# Autodesk Inventor assembly: ArmTrussMIR
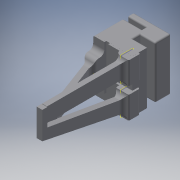
[picture p0: Inventor's stored thumbnail of the model, 180x180]
Saved by Autodesk Inventor 2018 (Build 220112000, 112)
## iProperties
Created: 2017-12-31
Part Number: ArmTrussMIR
Document SubType Name: Assembly
Designer: reide
Author: reide
## Documents named in this file (5)
- C:\Users\reide\OneDrive\Documents\Inventor\TSA\2018\Animatronics\Tortoise\arms\ArmTrussMIR.iam
- C:\Users\reide\OneDrive\Documents\Inventor\TSA\2018\Animatronics\Tortoise\arms\newShoulder_MIR.ipt
- C:\Users\reide\OneDrive\Documents\Inventor\TSA\2018\Animatronics\Tortoise\arms\straightBar_MIR.ipt
- C:\Users\reide\OneDrive\Documents\Inventor\TSA\2018\Animatronics\Tortoise\arms\AngleArm_MIR.ipt
- C:\Users\reide\OneDrive\Documents\Inventor\TSA\2018\Animatronics\Tortoise\arms\bottomARM_MIR.ipt
## Components (4 placed, 4 different names)
1. newShoulder_MIR:1
2. straightBar_MIR:1
3. AngleArm_MIR:1
4. bottomARM_MIR:1
## Relationships (9: Mate 5, Flush 4)
- [Mate]: newShoulder_MIR:1 ↔ straightBar_MIR:1
- [Mate]: newShoulder_MIR:1 ↔ straightBar_MIR:1
- [Flush]: newShoulder_MIR:1 ↔ straightBar_MIR:1
- [Mate]: newShoulder_MIR:1 ↔ AngleArm_MIR:1
- [Mate]: newShoulder_MIR:1 ↔ AngleArm_MIR:1
- [Flush]: newShoulder_MIR:1 ↔ AngleArm_MIR:1
- [Flush]: newShoulder_MIR:1 ↔ bottomARM_MIR:1
- [Flush]: newShoulder_MIR:1 ↔ bottomARM_MIR:1
- [Mate]: newShoulder_MIR:1 ↔ bottomARM_MIR:1
